# Autodesk Inventor assembly: 6P Sprocket
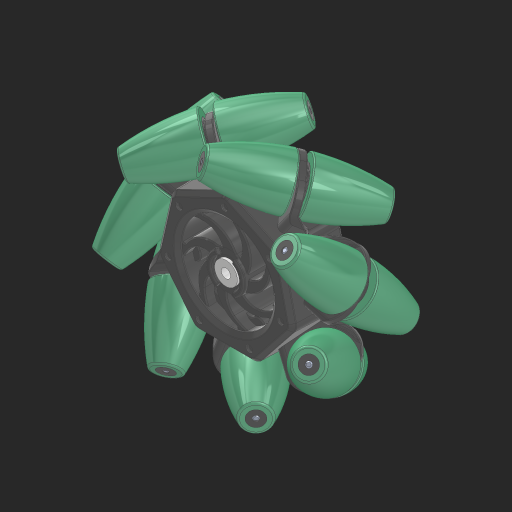
[picture p0: Inventor's stored thumbnail of the model, 512x512]
Saved by Autodesk Inventor 2023 (Build 270158000, 158)
## iProperties
Created: 2022-08-02
Part Number: 6P Sprocket
Document SubType Name: Assembly
Designer: ylu12
Author: ylu12
## Documents named in this file (4)
- C:\Users\ylu12\Documents\GitHub\VEX-CAD-Inventor\Motion\Wheels\Mecanum Wheel\4 Mecanum Left, Circle.iam
- C:\Users\ylu12\Documents\GitHub\VEX-CAD-Inventor\Motion\Insert Circle.ipt
- C:\Users\ylu12\Documents\GitHub\VEX-CAD-Inventor\Motion\Wheels\Reference Files\4 Mecanum Left.ipt
- C:\Users\ylu12\Documents\GitHub\VEX-CAD-Inventor\Motion\Wheels\Mecanum Wheel.iam
## Components (3 placed, 3 different names)
1. 4 Mecanum Left:1
2. Circle 1 — Mate:29, Angle:4, Symmetry:2
3. Circle 2 — Mate:26, Angle:3, Symmetry:2, Flush:11
## Relationships (9: Mate 4, Flush 2, Angle 2, Symmetry 1)
- [Flush]: 4 Mecanum Left:1
- [Mate]: 4 Mecanum Left:1
- [Mate]: 4 Mecanum Left:1
- Mate:26: Circle 2
- Mate:29: Circle 1
- Angle:3 (0 deg): Circle 2
- Angle:4 (0 deg): Circle 1
- Symmetry:2: Circle 1 ↔ Circle 2
- Flush:11 (12 mm): Circle 2
## Named parameters: Thickness = 12 mm
